# Autodesk Inventor assembly: blob_all
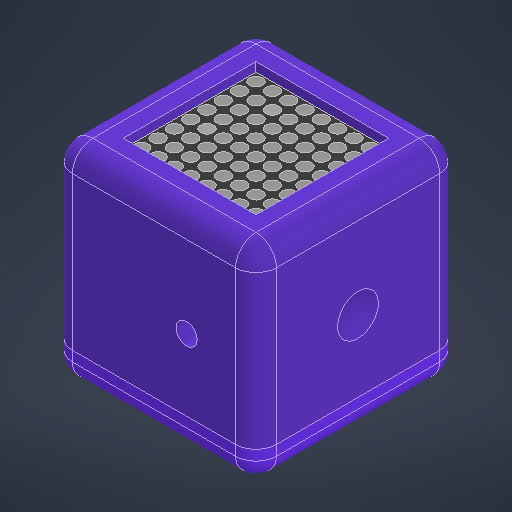
[picture p0: Inventor's stored thumbnail of the model, 512x512]
Saved by Autodesk Inventor 2026.2 (Build 302298000, 298)
## iProperties
Created: 2025-06-28
Part Number: blob_all
Document SubType Name: Assembly
Designer: micyg
Author: micyg
## Documents named in this file (7)
- D:\Projects\VirtualPets\VirtualBlob\Mechanical\blob_all.iam
- D:\Projects\VirtualPets\VirtualBlob\Mechanical\case1.ipt
- D:\Projects\VirtualPets\VirtualBlob\Mechanical\case2.ipt
- D:\Projects\VirtualPets\VirtualBlob\Mechanical\battery.ipt
- D:\Projects\VirtualPets\VirtualBlob\Mechanical\boards\MainBoard\mainboard_0_4_0\VirtualBlob_MainBoard_0.4.0\VirtualBlob_MainBoard_0.4.0.iam
- D:\Projects\VirtualPets\VirtualBlob\Mechanical\touchSpring.ipt
- D:\Projects\VirtualPets\VirtualBlob\Mechanical\matrix.iam
## Components (6 placed, 6 different names)
1. case1:1 — Mate:3, Mate:9, Mate:17, Mate:18, Mate:19, Mate:23, Mate:24, Mate:25, Mate:26, Mate:27
2. case2:1 — Mate:3, Mate:9, Mate:10, Mate:11, Mate:12, Mate:23
3. battery:1 — Mate:17, Mate:18, Mate:19, Mate:24
4. VirtualBlob_MainBoard_0.4.0:1 [sub-assembly] — Mate:10, Mate:11, Mate:12, Mate:14, Mate:15, Mate:16
5. touchSpring:1 — Mate:14, Mate:15, Mate:16
6. matrix:1 [sub-assembly] — Mate:25, Mate:26, Mate:27
## Relationships (16: Mate 16)
- Mate:3: case1:1 ↔ case2:1
- Mate:9: case1:1 ↔ case2:1
- Mate:10: case2:1 ↔ VirtualBlob_MainBoard_0.4.0:1
- Mate:11: case2:1 ↔ VirtualBlob_MainBoard_0.4.0:1
- Mate:12: case2:1 ↔ VirtualBlob_MainBoard_0.4.0:1
- Mate:14: VirtualBlob_MainBoard_0.4.0:1 ↔ touchSpring:1
- Mate:15: VirtualBlob_MainBoard_0.4.0:1 ↔ touchSpring:1
- Mate:16: VirtualBlob_MainBoard_0.4.0:1 ↔ touchSpring:1
- Mate:17: case1:1 ↔ battery:1
- Mate:18: case1:1 ↔ battery:1
- Mate:19: case1:1 ↔ battery:1
- Mate:23: case1:1 ↔ case2:1
- Mate:24 (4 mm): case1:1 ↔ battery:1
- Mate:25: case1:1 ↔ matrix:1
- Mate:26 (0.25 mm): case1:1 ↔ matrix:1
- Mate:27 (0.25 mm): case1:1 ↔ matrix:1
